# Autodesk Inventor assembly: Profile Endstop Assembly - XDirLimit
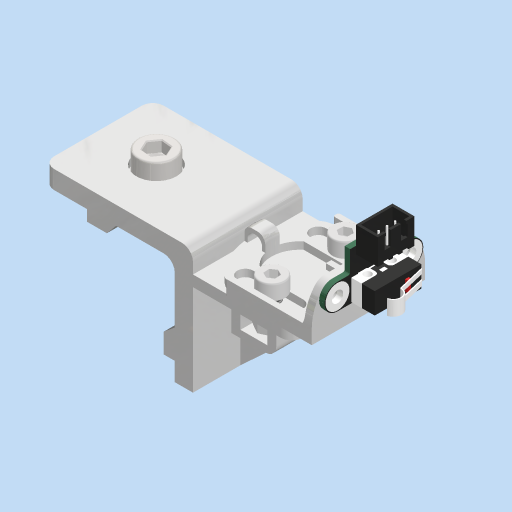
[picture p0: Inventor's stored thumbnail of the model, 512x512]
Saved by Autodesk Inventor 2023.2 (Build 272271000, 271)
## iProperties
Created: 2024-02-13
Part Number: Profile Endstop Assembly - XDirLimit
Document SubType Name: Assembly
Designer: Nils Bade
Author: Nils Bade
## Documents named in this file (8)
- C:\Users\nilsb\Documents\Inventor\Projektarbeit-Bade\RatRig_Bade\Profile Endstop Assembly - XDirLimit.iam
- C:\Users\nilsb\Documents\Inventor\Projektarbeit-Bade\RatRig_modified\Profile Endstop Mount.ipt
- C:\Users\nilsb\Documents\Inventor\Projektarbeit-Bade\RatRig_modified\T-NUT - DropIn 4040 SERIES - M6.ipt
- C:\Users\nilsb\Documents\Inventor\Projektarbeit-Bade\Schrauben\Cap Head Screw M6x12 v2.ipt
- C:\Users\nilsb\Documents\Inventor\Projektarbeit-Bade\RatRig_modified\X-Gantry Enstop Mount.ipt
- C:\Users\nilsb\Documents\Inventor\Projektarbeit-Bade\RatRig_modified\Endstop-Horizontal-RatRig.ipt
- C:\Users\nilsb\Documents\Inventor\Projektarbeit-Bade\Schrauben\Cap Head Screw M4x12 - DIN912.ipt
- C:\Users\nilsb\Documents\Inventor\Projektarbeit-Bade\RatRig_Standards\Hex Nut - M4 DIN934.ipt
## Components (9 placed, 7 different names)
1. Profile Endstop Mount:1 — Passend:1, Passend:2, Winkel:1, Passend:3, Passend:4, Passend:5, Passend:6, Passend:7, Passend:11, Passend:12, Passend:17, Passend:18, Winkel:2, Winkel:3, Fluchtend:1
2. T-NUT - DROP IN TYPE FOR 40 SERIES - M6:1 — Passend:1, Passend:2, Winkel:1
3. Cap Head Screw M6x12 v2:1 — Passend:3, Passend:4
4. X-Gantry Enstop Mount:1 — Passend:5, Passend:6, Passend:7, Passend:8, Passend:9, Passend:10, Passend:13, Passend:14, Fluchtend:1
5. Endstop-Horizontal-RatRig:1 — Passend:8, Passend:9, Passend:10
6. Cap Head Screw M4x12 - DIN912:1 — Passend:11, Passend:14, Passend:15
7. Cap Head Screw M4x12 - DIN912:2 — Passend:12, Passend:13, Passend:16
8. Hex Nut - M4 DIN934:1 — Passend:15, Passend:18, Winkel:2
9. Hex Nut - M4 DIN934:2 — Passend:16, Passend:17, Winkel:3
## Relationships (22: Mate 18, Angle 3, Flush 1)
- Passend:1 [Mate]: Profile Endstop Mount:1 ↔ T-NUT - DROP IN TYPE FOR 40 SERIES - M6:1
- Passend:2 [Mate] (4.5 mm): Profile Endstop Mount:1 ↔ T-NUT - DROP IN TYPE FOR 40 SERIES - M6:1
- Winkel:1 [Angle] (0 deg): Profile Endstop Mount:1 ↔ T-NUT - DROP IN TYPE FOR 40 SERIES - M6:1
- Passend:3 [Mate]: Profile Endstop Mount:1 ↔ Cap Head Screw M6x12 v2:1
- Passend:4 [Mate]: Profile Endstop Mount:1 ↔ Cap Head Screw M6x12 v2:1
- Passend:5 [Mate]: Profile Endstop Mount:1 ↔ X-Gantry Enstop Mount:1
- Passend:6 [Mate]: Profile Endstop Mount:1 ↔ X-Gantry Enstop Mount:1
- Passend:7 [Mate]: Profile Endstop Mount:1 ↔ X-Gantry Enstop Mount:1
- Passend:8 [Mate]: X-Gantry Enstop Mount:1 ↔ Endstop-Horizontal-RatRig:1
- Passend:9 [Mate]: X-Gantry Enstop Mount:1 ↔ Endstop-Horizontal-RatRig:1
- Passend:10 [Mate]: X-Gantry Enstop Mount:1 ↔ Endstop-Horizontal-RatRig:1
- Passend:11 [Mate]: Profile Endstop Mount:1 ↔ Cap Head Screw M4x12 - DIN912:1
- Passend:12 [Mate]: Profile Endstop Mount:1 ↔ Cap Head Screw M4x12 - DIN912:2
- Passend:13 [Mate]: X-Gantry Enstop Mount:1 ↔ Cap Head Screw M4x12 - DIN912:2
- Passend:14 [Mate]: X-Gantry Enstop Mount:1 ↔ Cap Head Screw M4x12 - DIN912:1
- Passend:15 [Mate]: Cap Head Screw M4x12 - DIN912:1 ↔ Hex Nut - M4 DIN934:1
- Passend:16 [Mate]: Cap Head Screw M4x12 - DIN912:2 ↔ Hex Nut - M4 DIN934:2
- Passend:17 [Mate]: Profile Endstop Mount:1 ↔ Hex Nut - M4 DIN934:2
- Passend:18 [Mate]: Profile Endstop Mount:1 ↔ Hex Nut - M4 DIN934:1
- Winkel:2 [Angle] (0 deg): Profile Endstop Mount:1 ↔ Hex Nut - M4 DIN934:1
- Winkel:3 [Angle] (0 deg): Profile Endstop Mount:1 ↔ Hex Nut - M4 DIN934:2
- Fluchtend:1 [Flush] (-6 mm): Profile Endstop Mount:1 ↔ X-Gantry Enstop Mount:1
